# Autodesk Inventor assembly: assembly_hoop
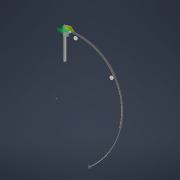
[picture p0: Inventor's stored thumbnail of the model, 180x180]
Saved by Autodesk Inventor 2021 (Build 250183000, 183)
## iProperties
Created: 2021-05-25
Part Number: assembly_hoop
Document SubType Name: Assembly
Designer: Watchdog
Author: Watchdog
## Documents named in this file (6)
- C:\Users\Watchdog\OneDrive - Flinders\Advn Mech Design Shared\6_Development\2_Design\inventor\assembly_hoop.iam
- C:\Users\Watchdog\OneDrive - Flinders\Advn Mech Design Shared\6_Development\2_Design\inventor\support\support_frameAssembly.iam
- C:\Users\Watchdog\OneDrive - Flinders\Advn Mech Design Shared\6_Development\2_Design\inventor\hoop_slider\hoops_sml_med_lrg.iam
- C:\Users\Watchdog\OneDrive - Flinders\Advn Mech Design Shared\6_Development\2_Design\inventor\support\reel\reelTab.ipt
- C:\Users\Watchdog\OneDrive - Flinders\Advn Mech Design Shared\6_Development\2_Design\inventor\support\reel\SKF_608.iam
- C:\Users\Watchdog\OneDrive - Flinders\Advn Mech Design Shared\6_Development\2_Design\inventor\support\reel\motorAssembly.iam
## Components (5 placed, 5 different names)
1. support_frameAssembly:1 [sub-assembly] — Flush:1, Flush:2, Mate:1, Mate:6, Mate:8, Mate:9, Mate:10, Mate:11, Mate:12, Mate:16
2. hoops_sml_med_lrg:1 [sub-assembly] — Mate:6, Mate:8, Mate:9
3. reelTab:1 — Mate:10, Mate:11, Mate:12, Mate:13, Flush:3
4. SKF_608:1 [sub-assembly] — Mate:13, Flush:3, Mate:17, Mate:18
5. motorAssembly:1 [sub-assembly] — Mate:16, Mate:17, Mate:18
## Relationships (14: Mate 11, Flush 3)
- Flush:1: support_frameAssembly:1
- Flush:2: support_frameAssembly:1
- Mate:1: support_frameAssembly:1
- Mate:6: support_frameAssembly:1 ↔ hoops_sml_med_lrg:1
- Mate:8: support_frameAssembly:1 ↔ hoops_sml_med_lrg:1
- Mate:9: support_frameAssembly:1 ↔ hoops_sml_med_lrg:1
- Mate:10: support_frameAssembly:1 ↔ reelTab:1
- Mate:11: support_frameAssembly:1 ↔ reelTab:1
- Mate:12: support_frameAssembly:1 ↔ reelTab:1
- Mate:13: reelTab:1 ↔ SKF_608:1
- Flush:3: reelTab:1 ↔ SKF_608:1
- Mate:16: support_frameAssembly:1 ↔ motorAssembly:1
- Mate:17: SKF_608:1 ↔ motorAssembly:1
- Mate:18: SKF_608:1 ↔ motorAssembly:1
